# Autodesk Inventor assembly: External Frame Assembly
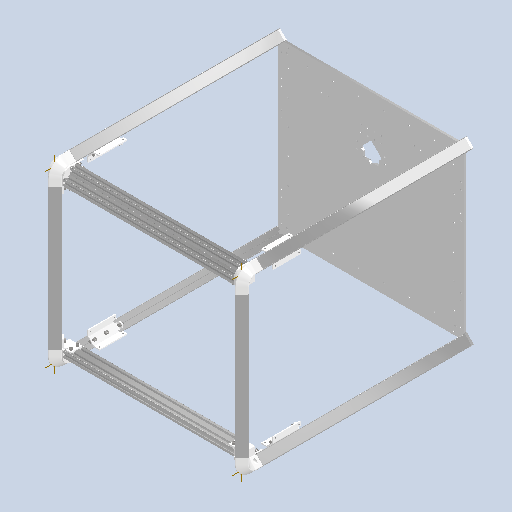
[picture p0: Inventor's stored thumbnail of the model, 512x512]
Saved by Autodesk Inventor 2024 (Build 280153000, 153)
## iProperties
Created: 2024-12-02
Part Number: External Frame Assembly
Document SubType Name: Assembly
Designer: Ishaan
Author: Ishaan
## Documents named in this file (14)
- E:\Projects\Axiom--IDEX-3D-Printer\CAD\08 - Side Panelling\External Frame Assembly.iam
- E:\Projects\Axiom--IDEX-3D-Printer\CAD\02 - Frame\Printer Base Plate RevII.ipt
- E:\Projects\Axiom--IDEX-3D-Printer\CAD\08 - Side Panelling\Exterior Frame Corner R2.ipt
- E:\Projects\Axiom--IDEX-3D-Printer\CAD\00 - COTS Components\3030 Frame Exterior Y Runners\HFSC6-3030-417.ipt
- E:\Projects\Axiom--IDEX-3D-Printer\CAD\00 - COTS Components\4040 Frame Exterior X Runners\HFS5-404020-505.ipt
- E:\Projects\Axiom--IDEX-3D-Printer\CAD\08 - Side Panelling\External Frame Corner Bracket.ipt
- E:\Projects\Axiom--IDEX-3D-Printer\CAD\08 - Side Panelling\External Frame Corner Bracket Mirror.ipt
- E:\Projects\Axiom--IDEX-3D-Printer\CAD\00 - COTS Components\Hardware\M5 T SLOT NUT.ipt
- E:\Projects\Axiom--IDEX-3D-Printer\CAD\00 - COTS Components\Hardware\SHCSM5x8.ipt
- E:\Projects\Axiom--IDEX-3D-Printer\CAD\00 - COTS Components\Hardware\SHCSM5x20.ipt
- E:\Projects\Axiom--IDEX-3D-Printer\CAD\00 - COTS Components\Hardware\M6 T SLOT NUT 3030.ipt
- E:\Projects\Axiom--IDEX-3D-Printer\CAD\08 - Side Panelling\Exterior Frame Gantry Brace.ipt
- E:\Projects\Axiom--IDEX-3D-Printer\CAD\00 - COTS Components\Hardware\SHCSM6x10.ipt
- E:\Projects\Axiom--IDEX-3D-Printer\CAD\00 - COTS Components\3030 External Frame Risers\HFSC6-3030-616.ipt
## Components (101 placed, 13 different names)
1. Printer Base Plate RevII:1
2. HFSC6-3030-616:1
3. HFSC6-3030-616:2
4. HFSC6-3030-616:3
5. HFSC6-3030-616:4
6. Exterior Frame Corner R2:1 — Mate:7, Mate:15, Insert:5, Insert:8, Insert:39, Insert:40
7. Exterior Frame Corner R2:2 — Mate:7, Mate:14, Mate:16, Angle:2, Insert:11, Insert:12, Insert:37, Insert:38
8. Exterior Frame Corner R2:3 — Mate:10, Mate:11, Mate:13, Insert:6, Insert:7, Insert:35, Insert:36
9. Exterior Frame Corner R2:4 — Mate:10, Angle:1, Mate:12, Insert:9, Insert:10, Insert:33, Insert:34
10. HFSC6-3030-417:1 — Mate:11, Angle:1, Mate:12, Mate:13, Mate:19, Mate:25
11. HFSC6-3030-417:2 — Mate:14, Mate:15, Mate:16, Angle:2, Mate:23, Mate:29
12. HFS5-404020-505:1 — Insert:5, Insert:6, Insert:7, Insert:8, Mate:18, Flush:5, Mate:20, Flush:6, Mate:28, Flush:10, Mate:30, Flush:11, Angle:11, Angle:12, Angle:13, Angle:14
13. HFS5-404020-505:2 — Insert:9, Insert:10, Insert:11, Insert:12, Mate:22, Flush:7, Mate:24, Flush:8, Mate:26, Flush:9, Mate:32, Flush:12, Angle:15, Angle:16, Angle:17, Angle:18, Flush:13, Flush:14
14. External Frame Corner Bracket:1 — Mate:18, Flush:5, Insert:30, Insert:55
15. External Frame Corner Bracket:2 — Mate:19, Mate:20, Flush:6, Insert:23, Insert:24, Insert:49
16. External Frame Corner Bracket:3 — Mate:22, Flush:7, Insert:27, Insert:28, Insert:47
17. External Frame Corner Bracket:4 — Mate:23, Mate:24, Flush:8, Insert:31, Insert:57
18. External Frame Corner Bracket Mirror:1 — Mate:29, Mate:30, Flush:11, Insert:29, Insert:56
19. External Frame Corner Bracket Mirror:2 — Mate:32, Flush:12, Insert:32, Insert:58
20. External Frame Corner Bracket Mirror:3 — Mate:28, Flush:10, Insert:21, Insert:22, Insert:50
21. External Frame Corner Bracket Mirror:4 — Mate:25, Mate:26, Flush:9, Insert:25, Insert:26, Insert:48
22. Exterior Frame Gantry Brace:1 — Flush:13, Flush:14, Flush:15, Flush:16, Flush:20, Insert:41, Insert:45, Insert:46, Insert:61
23. Exterior Frame Gantry Brace:2 — Flush:15, Flush:16, Flush:17, Flush:18, Insert:42, Insert:59, Insert:60, Insert:63
24. Exterior Frame Gantry Brace:3 — Flush:17, Flush:18, Flush:19, Flush:21, Insert:43, Insert:53, Insert:54, Insert:64
25. Exterior Frame Gantry Brace:4 — Flush:19, Flush:20, Flush:21, Insert:44, Insert:51, Insert:52, Insert:62
26. SHCSM5x8:17 — Insert:61
27. SHCSM5x8:18 — Insert:62
28. SHCSM5x8:19 — Insert:64
29. SHCSM5x8:20 — Insert:63
30. SHCSM6x10:1 — Insert:45
31. SHCSM6x10:2 — Insert:46
32. SHCSM6x10:3 — Insert:47
33. SHCSM6x10:4 — Insert:48
34. SHCSM6x10:5 — Insert:49
35. SHCSM6x10:6 — Insert:50
36. SHCSM6x10:7 — Insert:51
37. SHCSM6x10:8 — Insert:52
38. SHCSM6x10:9 — Insert:60
39. SHCSM6x10:10 — Insert:59
40. SHCSM6x10:11 — Insert:58
41. SHCSM6x10:12 — Insert:57
42. SHCSM6x10:13 — Insert:56
43. SHCSM6x10:14 — Insert:53
44. SHCSM6x10:15 — Insert:54
45. SHCSM6x10:16 — Insert:55
46. SHCSM5x20:1 — Insert:36
47. SHCSM5x20:2 — Insert:35
48. SHCSM5x20:3 — Insert:34
49. SHCSM5x20:4 — Insert:33
50. SHCSM5x20:5 — Insert:37
51. SHCSM5x20:6 — Insert:38
52. SHCSM5x20:7 — Insert:39
53. SHCSM5x20:8 — Insert:40
54. M6 T SLOT NUT 3030:1
55. M6 T SLOT NUT 3030:2
56. M6 T SLOT NUT 3030:3
57. M6 T SLOT NUT 3030:4
58. M6 T SLOT NUT 3030:5
59. M6 T SLOT NUT 3030:6
60. M6 T SLOT NUT 3030:7
61. M6 T SLOT NUT 3030:8
62. M6 T SLOT NUT 3030:9 — Insert:41
63. M6 T SLOT NUT 3030:10
64. M6 T SLOT NUT 3030:11 — Insert:42
65. M6 T SLOT NUT 3030:12
66. M6 T SLOT NUT 3030:13 — Insert:43
67. M6 T SLOT NUT 3030:14
68. M6 T SLOT NUT 3030:15 — Insert:44
69. M6 T SLOT NUT 3030:16
70. SHCSM5x8:1 — Insert:29
71. SHCSM5x8:2
72. SHCSM5x8:3
73. SHCSM5x8:4
74. SHCSM5x8:5 — Insert:30
75. SHCSM5x8:6
76. SHCSM5x8:7
77. SHCSM5x8:8
78. SHCSM5x8:9 — Insert:31
79. SHCSM5x8:11
80. SHCSM5x8:12
81. SHCSM5x8:13
82. SHCSM5x8:10 — Insert:32
83. SHCSM5x8:14
84. SHCSM5x8:15
85. SHCSM5x8:16
86. M5 T SLOT NUT:5 — Insert:28, Angle:15
87. M5 T SLOT NUT:6 — Insert:27, Angle:16
88. M5 T SLOT NUT:8 — Insert:25, Angle:17
89. M5 T SLOT NUT:7 — Insert:26, Angle:18
90. M5 T SLOT NUT:9
91. M5 T SLOT NUT:10
92. M5 T SLOT NUT:11
93. M5 T SLOT NUT:12
94. M5 T SLOT NUT:4 — Insert:24, Angle:13
95. M5 T SLOT NUT:3 — Insert:23, Angle:14
96. M5 T SLOT NUT:2 — Insert:22, Angle:12
97. M5 T SLOT NUT:1 — Insert:21, Angle:11
98. M5 T SLOT NUT:13
99. M5 T SLOT NUT:14
100. M5 T SLOT NUT:15
101. M5 T SLOT NUT:16
## Component patterns: (2 elements, first: M6 T SLOT NUT 3030:9), (2 elements, first: M6 T SLOT NUT 3030:11), (2 elements, first: M6 T SLOT NUT 3030:13), (2 elements, first: M6 T SLOT NUT 3030:15), (4 elements, first: SHCSM5x8:1), (4 elements, first: SHCSM5x8:5), (4 elements, first: SHCSM5x8:9), (4 elements, first: SHCSM5x8:10), (2 elements, first: M5 T SLOT NUT:5 + M5 T SLOT NUT:6 + M5 T SLOT NUT:8 + M5 T SLOT NUT:7), (2 elements, first: M5 T SLOT NUT:4 + M5 T SLOT NUT:3 + M5 T SLOT NUT:2 + M5 T SLOT NUT:1)
## Relationships (143: Insert 64, Mate 36, Angle 22, Flush 21)
- [Insert]: Printer Base Plate RevII:1 ↔ HFSC6-3030-616:1
- [Insert]: Printer Base Plate RevII:1 ↔ HFSC6-3030-616:2
- [Insert]: Printer Base Plate RevII:1 ↔ HFSC6-3030-616:3
- [Insert]: Printer Base Plate RevII:1 ↔ HFSC6-3030-616:4
- [Flush]: Printer Base Plate RevII:1 ↔ HFSC6-3030-616:2
- [Flush]: Printer Base Plate RevII:1 ↔ HFSC6-3030-616:1
- [Flush]: Printer Base Plate RevII:1 ↔ HFSC6-3030-616:3
- [Flush]: Printer Base Plate RevII:1 ↔ HFSC6-3030-616:4
- [Mate]: HFSC6-3030-616:1 ↔ Exterior Frame Corner R2:1
- [Mate] (0.2 mm): HFSC6-3030-616:1 ↔ Exterior Frame Corner R2:1
- [Mate]: HFSC6-3030-616:4 ↔ Exterior Frame Corner R2:4
- [Mate] (0.2 mm): HFSC6-3030-616:4 ↔ Exterior Frame Corner R2:4
- [Mate]: HFSC6-3030-616:3 ↔ Exterior Frame Corner R2:2
- [Mate] (0.2 mm): HFSC6-3030-616:3 ↔ Exterior Frame Corner R2:2
- Mate:7: Exterior Frame Corner R2:1 ↔ Exterior Frame Corner R2:2
- [Mate]: HFSC6-3030-616:2 ↔ Exterior Frame Corner R2:3
- [Mate] (0.2 mm): HFSC6-3030-616:2 ↔ Exterior Frame Corner R2:3
- Mate:10: Exterior Frame Corner R2:3 ↔ Exterior Frame Corner R2:4
- Mate:11: Exterior Frame Corner R2:3 ↔ HFSC6-3030-417:1
- Angle:1 (0 deg): Exterior Frame Corner R2:4 ↔ HFSC6-3030-417:1
- Mate:12 (0.2 mm): Exterior Frame Corner R2:4 ↔ HFSC6-3030-417:1
- Mate:13 (0.2 mm): Exterior Frame Corner R2:3 ↔ HFSC6-3030-417:1
- Mate:14: Exterior Frame Corner R2:2 ↔ HFSC6-3030-417:2
- Mate:15 (0.2 mm): Exterior Frame Corner R2:1 ↔ HFSC6-3030-417:2
- Mate:16 (0.2 mm): Exterior Frame Corner R2:2 ↔ HFSC6-3030-417:2
- Angle:2 (0 deg): Exterior Frame Corner R2:2 ↔ HFSC6-3030-417:2
- Insert:5 (0.2 mm): Exterior Frame Corner R2:1 ↔ HFS5-404020-505:1
- Insert:6 (0.2 mm): Exterior Frame Corner R2:3 ↔ HFS5-404020-505:1
- Insert:7 (0.2 mm): Exterior Frame Corner R2:3 ↔ HFS5-404020-505:1
- Insert:8 (0.2 mm): Exterior Frame Corner R2:1 ↔ HFS5-404020-505:1
- Insert:9 (0.2 mm): Exterior Frame Corner R2:4 ↔ HFS5-404020-505:2
- Insert:10 (0.2 mm): Exterior Frame Corner R2:4 ↔ HFS5-404020-505:2
- Insert:11 (0.2 mm): Exterior Frame Corner R2:2 ↔ HFS5-404020-505:2
- Insert:12 (0.2 mm): Exterior Frame Corner R2:2 ↔ HFS5-404020-505:2
- [Mate]: HFSC6-3030-616:1 ↔ External Frame Corner Bracket:1
- Mate:18: HFS5-404020-505:1 ↔ External Frame Corner Bracket:1
- Flush:5 (-2.5 mm): HFS5-404020-505:1 ↔ External Frame Corner Bracket:1
- Mate:19: HFSC6-3030-417:1 ↔ External Frame Corner Bracket:2
- Mate:20: HFS5-404020-505:1 ↔ External Frame Corner Bracket:2
- Flush:6 (-2.5 mm): HFS5-404020-505:1 ↔ External Frame Corner Bracket:2
- [Mate]: HFSC6-3030-616:4 ↔ External Frame Corner Bracket:3
- Mate:22: HFS5-404020-505:2 ↔ External Frame Corner Bracket:3
- Flush:7 (-2.5 mm): HFS5-404020-505:2 ↔ External Frame Corner Bracket:3
- Mate:23: HFSC6-3030-417:2 ↔ External Frame Corner Bracket:4
- Mate:24: HFS5-404020-505:2 ↔ External Frame Corner Bracket:4
- Flush:8 (-2.5 mm): HFS5-404020-505:2 ↔ External Frame Corner Bracket:4
- Mate:25: HFSC6-3030-417:1 ↔ External Frame Corner Bracket Mirror:4
- Mate:26: HFS5-404020-505:2 ↔ External Frame Corner Bracket Mirror:4
- Flush:9 (-2.5 mm): HFS5-404020-505:2 ↔ External Frame Corner Bracket Mirror:4
- [Mate]: HFSC6-3030-616:2 ↔ External Frame Corner Bracket Mirror:3
- Mate:28: HFS5-404020-505:1 ↔ External Frame Corner Bracket Mirror:3
- Flush:10 (-2.5 mm): HFS5-404020-505:1 ↔ External Frame Corner Bracket Mirror:3
- Mate:29: HFSC6-3030-417:2 ↔ External Frame Corner Bracket Mirror:1
- Mate:30: HFS5-404020-505:1 ↔ External Frame Corner Bracket Mirror:1
- Flush:11 (-2.5 mm): HFS5-404020-505:1 ↔ External Frame Corner Bracket Mirror:1
- [Mate]: HFSC6-3030-616:3 ↔ External Frame Corner Bracket Mirror:2
- Mate:32: HFS5-404020-505:2 ↔ External Frame Corner Bracket Mirror:2
- Flush:12 (-2.5 mm): HFS5-404020-505:2 ↔ External Frame Corner Bracket Mirror:2
- [Insert]: External Frame Corner Bracket Mirror:1 ↔ M6 T SLOT NUT 3030:8
- [Angle] (0 deg): External Frame Corner Bracket Mirror:1 ↔ M6 T SLOT NUT 3030:8
- [Insert]: External Frame Corner Bracket:1 ↔ M6 T SLOT NUT 3030:7
- [Angle] (0 deg): External Frame Corner Bracket:1 ↔ M6 T SLOT NUT 3030:7
- [Insert]: External Frame Corner Bracket:2 ↔ M6 T SLOT NUT 3030:6
- [Angle] (0 deg): External Frame Corner Bracket:2 ↔ M6 T SLOT NUT 3030:6
- [Insert]: External Frame Corner Bracket Mirror:4 ↔ M6 T SLOT NUT 3030:5
- [Angle] (0 deg): External Frame Corner Bracket Mirror:4 ↔ M6 T SLOT NUT 3030:5
- [Insert]: External Frame Corner Bracket:4 ↔ M6 T SLOT NUT 3030:2
- [Angle] (0 deg): External Frame Corner Bracket:4 ↔ M6 T SLOT NUT 3030:2
- [Insert]: External Frame Corner Bracket Mirror:2 ↔ M6 T SLOT NUT 3030:1
- [Angle] (0 deg): External Frame Corner Bracket Mirror:2 ↔ M6 T SLOT NUT 3030:1
- [Insert]: External Frame Corner Bracket:3 ↔ M6 T SLOT NUT 3030:4
- [Angle] (0 deg): External Frame Corner Bracket:3 ↔ M6 T SLOT NUT 3030:4
- [Insert]: External Frame Corner Bracket Mirror:3 ↔ M6 T SLOT NUT 3030:3
- [Angle] (0 deg): External Frame Corner Bracket Mirror:3 ↔ M6 T SLOT NUT 3030:3
- Insert:21 (2 mm): External Frame Corner Bracket Mirror:3 ↔ M5 T SLOT NUT:1
- Angle:11 (0 deg): HFS5-404020-505:1 ↔ M5 T SLOT NUT:1
- Insert:22 (2 mm): External Frame Corner Bracket Mirror:3 ↔ M5 T SLOT NUT:2
- Angle:12 (0 deg): HFS5-404020-505:1 ↔ M5 T SLOT NUT:2
- Insert:23 (2 mm): External Frame Corner Bracket:2 ↔ M5 T SLOT NUT:3
- Insert:24 (2 mm): External Frame Corner Bracket:2 ↔ M5 T SLOT NUT:4
- Angle:13 (0 deg): HFS5-404020-505:1 ↔ M5 T SLOT NUT:4
- Angle:14 (0 deg): HFS5-404020-505:1 ↔ M5 T SLOT NUT:3
- Insert:25 (2 mm): External Frame Corner Bracket Mirror:4 ↔ M5 T SLOT NUT:8
- Insert:26 (2 mm): External Frame Corner Bracket Mirror:4 ↔ M5 T SLOT NUT:7
- Insert:27 (2 mm): External Frame Corner Bracket:3 ↔ M5 T SLOT NUT:6
- Insert:28 (2 mm): External Frame Corner Bracket:3 ↔ M5 T SLOT NUT:5
- Angle:15 (0 deg): HFS5-404020-505:2 ↔ M5 T SLOT NUT:5
- Angle:16 (0 deg): HFS5-404020-505:2 ↔ M5 T SLOT NUT:6
- Angle:17 (0 deg): HFS5-404020-505:2 ↔ M5 T SLOT NUT:8
- Angle:18 (0 deg): HFS5-404020-505:2 ↔ M5 T SLOT NUT:7
- Insert:29: External Frame Corner Bracket Mirror:1 ↔ SHCSM5x8:1
- Insert:30: External Frame Corner Bracket:1 ↔ SHCSM5x8:5
- Insert:31: External Frame Corner Bracket:4 ↔ SHCSM5x8:9
- Insert:32: External Frame Corner Bracket Mirror:2 ↔ SHCSM5x8:10
- Insert:33: Exterior Frame Corner R2:4 ↔ SHCSM5x20:4
- Insert:34: Exterior Frame Corner R2:4 ↔ SHCSM5x20:3
- Insert:35: Exterior Frame Corner R2:3 ↔ SHCSM5x20:2
- Insert:36: Exterior Frame Corner R2:3 ↔ SHCSM5x20:1
- Insert:37: Exterior Frame Corner R2:2 ↔ SHCSM5x20:5
- Insert:38: Exterior Frame Corner R2:2 ↔ SHCSM5x20:6
- Insert:39: Exterior Frame Corner R2:1 ↔ SHCSM5x20:7
- Insert:40: Exterior Frame Corner R2:1 ↔ SHCSM5x20:8
- [Mate]: HFSC6-3030-616:4 ↔ Exterior Frame Gantry Brace:1
- Flush:13: HFS5-404020-505:2 ↔ Exterior Frame Gantry Brace:1
- Flush:14 (136.15 mm): HFS5-404020-505:2 ↔ Exterior Frame Gantry Brace:1
- [Mate]: HFSC6-3030-616:3 ↔ Exterior Frame Gantry Brace:2
- Flush:15: Exterior Frame Gantry Brace:1 ↔ Exterior Frame Gantry Brace:2
- Flush:16: Exterior Frame Gantry Brace:1 ↔ Exterior Frame Gantry Brace:2
- [Mate]: HFSC6-3030-616:1 ↔ Exterior Frame Gantry Brace:3
- Flush:17: Exterior Frame Gantry Brace:2 ↔ Exterior Frame Gantry Brace:3
- Flush:18: Exterior Frame Gantry Brace:2 ↔ Exterior Frame Gantry Brace:3
- [Mate]: HFSC6-3030-616:2 ↔ Exterior Frame Gantry Brace:4
- Flush:19: Exterior Frame Gantry Brace:3 ↔ Exterior Frame Gantry Brace:4
- Flush:20: Exterior Frame Gantry Brace:1 ↔ Exterior Frame Gantry Brace:4
- Flush:21: Exterior Frame Gantry Brace:3 ↔ Exterior Frame Gantry Brace:4
- Insert:41: Exterior Frame Gantry Brace:1 ↔ M6 T SLOT NUT 3030:9
- [Angle] (0 deg): HFSC6-3030-616:4 ↔ M6 T SLOT NUT 3030:9
- Insert:42: Exterior Frame Gantry Brace:2 ↔ M6 T SLOT NUT 3030:11
- [Angle] (0 deg): HFSC6-3030-616:3 ↔ M6 T SLOT NUT 3030:11
- Insert:43: Exterior Frame Gantry Brace:3 ↔ M6 T SLOT NUT 3030:13
- [Angle] (0 deg): HFSC6-3030-616:1 ↔ M6 T SLOT NUT 3030:13
- Insert:44: Exterior Frame Gantry Brace:4 ↔ M6 T SLOT NUT 3030:15
- [Angle] (0 deg): HFSC6-3030-616:2 ↔ M6 T SLOT NUT 3030:15
- Insert:45: Exterior Frame Gantry Brace:1 ↔ SHCSM6x10:1
- Insert:46: Exterior Frame Gantry Brace:1 ↔ SHCSM6x10:2
- Insert:47: External Frame Corner Bracket:3 ↔ SHCSM6x10:3
- Insert:48: External Frame Corner Bracket Mirror:4 ↔ SHCSM6x10:4
- Insert:49: External Frame Corner Bracket:2 ↔ SHCSM6x10:5
- Insert:50: External Frame Corner Bracket Mirror:3 ↔ SHCSM6x10:6
- Insert:51: Exterior Frame Gantry Brace:4 ↔ SHCSM6x10:7
- Insert:52: Exterior Frame Gantry Brace:4 ↔ SHCSM6x10:8
- Insert:53: Exterior Frame Gantry Brace:3 ↔ SHCSM6x10:14
- Insert:54: Exterior Frame Gantry Brace:3 ↔ SHCSM6x10:15
- Insert:55: External Frame Corner Bracket:1 ↔ SHCSM6x10:16
- Insert:56: External Frame Corner Bracket Mirror:1 ↔ SHCSM6x10:13
- Insert:57: External Frame Corner Bracket:4 ↔ SHCSM6x10:12
- Insert:58: External Frame Corner Bracket Mirror:2 ↔ SHCSM6x10:11
- Insert:59: Exterior Frame Gantry Brace:2 ↔ SHCSM6x10:10
- Insert:60: Exterior Frame Gantry Brace:2 ↔ SHCSM6x10:9
- Insert:61: Exterior Frame Gantry Brace:1 ↔ SHCSM5x8:17
- Insert:62: Exterior Frame Gantry Brace:4 ↔ SHCSM5x8:18
- Insert:63: Exterior Frame Gantry Brace:2 ↔ SHCSM5x8:20
- Insert:64: Exterior Frame Gantry Brace:3 ↔ SHCSM5x8:19
